# Autodesk Inventor assembly: Robot3rdYear
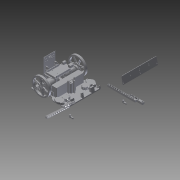
[picture p0: Inventor's stored thumbnail of the model, 180x180]
Saved by Autodesk Inventor 2011 SP2 (Build 150309200, 309)
## iProperties
Created: 2015-10-15
Part Number: Robot3rdYear
Document SubType Name: Assembly
Designer: Ernest
Author: Ernest
## Documents named in this file (17)
- D:\Inventor\Sumobot_3rd_Year\Robot3rdYear.iam
- D:\Inventor\Sumobot_3rd_Year\Cage.ipt
- D:\Inventor\Sumobot_3rd_Year\ArduinoMega.ipt
- D:\Inventor\Sumobot_3rd_Year\Battery9V.ipt
- D:\Inventor\Sumobot_3rd_Year\LineSensor.ipt
- D:\Inventor\Sumobot_3rd_Year\LiPoBattery.ipt
- D:\Inventor\Sumobot_3rd_Year\Motor12V.ipt
- D:\Inventor\Sumobot_3rd_Year\MotorDriver.ipt
- D:\Inventor\Sumobot_3rd_Year\Wheel90mm.ipt
- D:\Inventor\Sumobot_3rd_Year\Ball_and_Socket.ipt
- D:\Inventor\Sumobot_3rd_Year\MicroServo_Motor.ipt
- D:\Inventor\Sumobot_3rd_Year\Servo_Arm.ipt
- D:\Inventor\Sumobot_3rd_Year\Chassis.ipt
- D:\Inventor\Sumobot_3rd_Year\Robot_ARM_LEFT.ipt
- D:\Inventor\Sumobot_3rd_Year\Robot_ARM_RIGHT.ipt
- D:\Inventor\Sumobot_3rd_Year\Robot_ARM_Pivot.ipt
- D:\Inventor\Sumobot_3rd_Year\Front_Plate.ipt
## Components (25 placed, 16 different names)
1. Cage:1
2. ArduinoMega:1 — Mate:20, Mate:21, Flush:7
3. Battery9V:1 — Mate:31, Mate:46, Mate:47
4. LineSensor:1 — Mate:22, Mate:23, Flush:5
5. LineSensor:2 — Flush:6, Mate:24, Mate:25
6. LineSensor:3 — Mate:42, Mate:43, Flush:13
7. LineSensor:4 — Flush:12, Mate:37, Mate:38
8. LiPoBattery:1 — Mate:28, Mate:29, Mate:30
9. Motor12V:1 — Mate:4, Mate:7, Mate:8, Mate:9, Mate:12, Mate:13
10. Motor12V:2 — Mate:3, Mate:5, Mate:6, Mate:10, Mate:11, Mate:14
11. MotorDriver:1 — Mate:15, Mate:16, Mate:17
12. Wheel90mm:1 — Mate:12, Mate:13
13. Wheel90mm:2 — Mate:11, Mate:14
14. Ball_and_Socket:1 — Tangent:2, Mate:34, Mate:35
15. Ball_and_Socket:2 — Tangent:1, Angle:2, Mate:32, Mate:33, Mate:44, Mate:45
16. MicroServo_Motor:1 — Mate:18, Flush:2, Mate:26, Mate:48
17. MicroServo_Motor:2 — Mate:19, Flush:3, Mate:27, Mate:49
18. Servo_Arm:1 — Mate:19, Flush:3, Flush:11, Mate:41
19. Servo_Arm:2 — Mate:18, Flush:2, Mate:36, Mate:50
20. Chassis:1 — Mate:1, Mate:2, Flush:1, Mate:3, Mate:4, Mate:5, Mate:6, Mate:7, Mate:8, Mate:9, Mate:10, Mate:15, Mate:16, Mate:17, Mate:20, Mate:21, Mate:22, Mate:23, Flush:5, Flush:6, Mate:24, Mate:25, Mate:26, Mate:27, Angle:2, Mate:28, Mate:29, Mate:30, Mate:31, Flush:7, Flush:11, Flush:12, Mate:32, Mate:33, Mate:34, Mate:35, Mate:36, Mate:37, Mate:38, Mate:41, Mate:42, Mate:43, Flush:13, Mate:44, Mate:45, Mate:46, Mate:47, Mate:48, Mate:49
21. Robot_ARM_LEFT:1
22. Robot_ARM_RIGHT:1 — Mate:50
23. Robot_ARM_Pivot:1
24. Robot_ARM_Pivot:2
25. Front_Plate:1
## Relationships (60: Mate 48, Flush 9, Tangent 2, Angle 1)
- Mate:1 (3 mm): Chassis:1
- Mate:2: Chassis:1
- Flush:1 (69 mm): Chassis:1
- Mate:3: Motor12V:2 ↔ Chassis:1
- Mate:4: Motor12V:1 ↔ Chassis:1
- Mate:5: Motor12V:2 ↔ Chassis:1
- Mate:6: Motor12V:2 ↔ Chassis:1
- Mate:7: Motor12V:1 ↔ Chassis:1
- Mate:8: Motor12V:1 ↔ Chassis:1
- Mate:9: Motor12V:1 ↔ Chassis:1
- Mate:10: Motor12V:2 ↔ Chassis:1
- Mate:11: Motor12V:2 ↔ Wheel90mm:2
- Mate:12: Motor12V:1 ↔ Wheel90mm:1
- Mate:13: Motor12V:1 ↔ Wheel90mm:1
- Mate:14: Motor12V:2 ↔ Wheel90mm:2
- Mate:15: MotorDriver:1 ↔ Chassis:1
- Mate:16: MotorDriver:1 ↔ Chassis:1
- Mate:17: MotorDriver:1 ↔ Chassis:1
- Mate:18: MicroServo_Motor:1 ↔ Servo_Arm:2
- Flush:2 (5.7 mm): MicroServo_Motor:1 ↔ Servo_Arm:2
- Mate:19: MicroServo_Motor:2 ↔ Servo_Arm:1
- Flush:3 (5.7 mm): MicroServo_Motor:2 ↔ Servo_Arm:1
- Mate:20 (15.314 mm): ArduinoMega:1 ↔ Chassis:1
- Mate:21 (58 mm): ArduinoMega:1 ↔ Chassis:1
- Mate:22: LineSensor:1 ↔ Chassis:1
- Mate:23: LineSensor:1 ↔ Chassis:1
- Flush:5: LineSensor:1 ↔ Chassis:1
- Flush:6: LineSensor:2 ↔ Chassis:1
- Mate:24: LineSensor:2 ↔ Chassis:1
- Mate:25: LineSensor:2 ↔ Chassis:1
- Mate:26: MicroServo_Motor:1 ↔ Chassis:1
- Mate:27: MicroServo_Motor:2 ↔ Chassis:1
- Tangent:1: Ball_and_Socket:2
- Tangent:2: Ball_and_Socket:1
- Angle:2 (0 deg): Ball_and_Socket:2 ↔ Chassis:1
- Mate:28: LiPoBattery:1 ↔ Chassis:1
- Mate:29: LiPoBattery:1 ↔ Chassis:1
- Mate:30: LiPoBattery:1 ↔ Chassis:1
- Mate:31: Battery9V:1 ↔ Chassis:1
- Flush:7 (1.004 mm): ArduinoMega:1 ↔ Chassis:1
- Flush:11: Servo_Arm:1 ↔ Chassis:1
- Flush:12: LineSensor:4 ↔ Chassis:1
- Mate:32: Ball_and_Socket:2 ↔ Chassis:1
- Mate:33: Ball_and_Socket:2 ↔ Chassis:1
- Mate:34: Ball_and_Socket:1 ↔ Chassis:1
- Mate:35: Ball_and_Socket:1 ↔ Chassis:1
- Mate:36: Servo_Arm:2 ↔ Chassis:1
- Mate:37: LineSensor:4 ↔ Chassis:1
- Mate:38: LineSensor:4 ↔ Chassis:1
- Mate:41: Servo_Arm:1 ↔ Chassis:1
- Mate:42: LineSensor:3 ↔ Chassis:1
- Mate:43: LineSensor:3 ↔ Chassis:1
- Flush:13: LineSensor:3 ↔ Chassis:1
- Mate:44: Ball_and_Socket:2 ↔ Chassis:1
- Mate:45: Ball_and_Socket:2 ↔ Chassis:1
- Mate:46: Battery9V:1 ↔ Chassis:1
- Mate:47: Battery9V:1 ↔ Chassis:1
- Mate:48: MicroServo_Motor:1 ↔ Chassis:1
- Mate:49: MicroServo_Motor:2 ↔ Chassis:1
- Mate:50: Servo_Arm:2 ↔ Robot_ARM_RIGHT:1
